# Autodesk Inventor assembly: BD Drill motor assembly
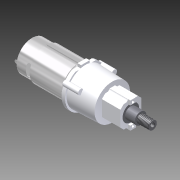
[picture p0: Inventor's stored thumbnail of the model, 180x180]
Saved by Autodesk Inventor 2012 (Build 160160000, 160)
## iProperties
Created: 2012-06-30
Part Number: BD Drill motor assembly
Document SubType Name: Assembly
Designer: Bruce
Author: Bruce
## Documents named in this file (5)
- C:\Users\FIRST\Dropbox\Inventor Design Project Files\Independent Swerves\Imported Components\BD Drill motor assembly.iam
- C:\Users\FIRST\Dropbox\Inventor Design Project Files\Independent Swerves\Imported Components\Gear housing BD drill motor.ipt
- C:\Users\FIRST\Dropbox\Inventor Design Project Files\Independent Swerves\Imported Components\FisherPriceMotor 550 motor.ipt
- C:\Users\FIRST\Dropbox\Inventor Design Project Files\Independent Swerves\Imported Components\Gear housing shaft BD drill motor.ipt
- C:\Users\FIRST\Dropbox\Inventor Design Project Files\Independent Swerves\Imported Components\Bearing BD drill motor shaft.ipt
## Components (4 placed, 4 different names)
1. Gear housing BD drill motor:1 — Mate:1, Flush:1, Mate:2, Mate:3, Flush:2
2. FisherPriceMotor 550 motor:1 — Mate:2, Mate:3
3. Gear housing shaft BD drill motor:1 — Mate:1, Flush:1, Mate:4
4. Bearing BD drill motor shaft:1 — Mate:4, Flush:2
## Relationships (6: Mate 4, Flush 2)
- Mate:1: Gear housing BD drill motor:1 ↔ Gear housing shaft BD drill motor:1
- Flush:1 (11.176 mm): Gear housing BD drill motor:1 ↔ Gear housing shaft BD drill motor:1
- Mate:2: Gear housing BD drill motor:1 ↔ FisherPriceMotor 550 motor:1
- Mate:3: Gear housing BD drill motor:1 ↔ FisherPriceMotor 550 motor:1
- Mate:4: Gear housing shaft BD drill motor:1 ↔ Bearing BD drill motor shaft:1
- Flush:2: Gear housing BD drill motor:1 ↔ Bearing BD drill motor shaft:1
